# Autodesk Inventor assembly: Assembly1
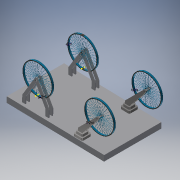
[picture p0: Inventor's stored thumbnail of the model, 180x180]
Saved by Autodesk Inventor 2018 (Build 220112000, 112)
## iProperties
Created: 2021-12-08
Part Number: Assembly1
Document SubType Name: Assembly
Designer: cs1190490
Author: cs1190490
## Documents named in this file (5)
- \\netapp1.iitd.ernet.in\homes\cse\btech\cs1190490\Windows\My Documents\Assembly1.iam
- \\netapp1.iitd.ernet.in\homes\cse\btech\cs1190490\Windows\Desktop\copy\Plate2.ipt
- \\netapp1.iitd.ernet.in\homes\cse\btech\cs1190490\Windows\Desktop\New folder\20 inch wheel.ipt
- \\netapp1.iitd.ernet.in\homes\cse\btech\cs1190490\Windows\My Documents\top.ipt
- \\netapp1.iitd.ernet.in\homes\cse\btech\cs1190490\Windows\My Documents\tri.ipt
## Components (9 placed, 4 different names)
1. Plate2:1 — Flush:1, Insert:1, Mate:1
2. 20 inch wheel:1 — Insert:1
3. top:1 — Flush:1, Mate:1, Mate:2, Mate:3, Mate:4, Mate:5, Mate:6, Mate:7
4. Plate2:2 — Mate:2, Mate:3, Insert:2
5. 20 inch wheel:2 — Insert:2
6. tri:1 — Mate:4, Mate:5, Insert:3, Mate:6
7. 20 inch wheel:3 — Insert:3
8. tri:2 — Mate:7, Mate:8
9. 20 inch wheel:4 — Mate:8
## Relationships (12: Mate 8, Insert 3, Flush 1)
- Flush:1 (50 mm): Plate2:1 ↔ top:1
- Insert:1 (-90 mm): Plate2:1 ↔ 20 inch wheel:1
- Mate:1: Plate2:1 ↔ top:1
- Mate:2: top:1 ↔ Plate2:2
- Mate:3 (-170 mm): top:1 ↔ Plate2:2
- Insert:2: Plate2:2 ↔ 20 inch wheel:2
- Mate:4: top:1 ↔ tri:1
- Mate:5 (-130 mm): top:1 ↔ tri:1
- Insert:3: tri:1 ↔ 20 inch wheel:3
- Mate:6: top:1 ↔ tri:1
- Mate:7: top:1 ↔ tri:2
- Mate:8: tri:2 ↔ 20 inch wheel:4
